# Autodesk Inventor assembly: Gearbox Assembly
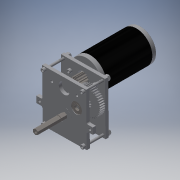
[picture p0: Inventor's stored thumbnail of the model, 180x180]
Saved by Autodesk Inventor 2018 (Build 220112000, 112)
## iProperties
Created: 2019-01-19
Part Number: Gearbox Assembly
Description: STEP AP203
Document SubType Name: Assembly
Designer: maste
Sending System: SolidWorks 2018
Preprocessor: SwSTEP 2.0
Title: Gear_Box.STEP
Revision Number: ANY
## Documents named in this file (17)
- C:\Users\s-2512711\Desktop\Github\2019CAD\Drivebase but Calvin is a mad man\Gearbox Assembly.iam
- C:\Users\s-2512711\Desktop\Github\2019CAD\Drivebase but Calvin is a mad man\CIM_Motor_217-2000.ipt
- C:\Users\s-2512711\Desktop\Github\2019CAD\Drivebase but Calvin is a mad man\12t_Steel_Spur_Gear_20_DP_CIM_Motor_217-3099.ipt
- C:\Users\s-2512711\Desktop\Github\2019CAD\Drivebase but Calvin is a mad man\14t_Steel_Spur_Gear_20_DP_3_8_Hex_Bore_217-3100.step.ipt
- C:\Users\s-2512711\Desktop\Github\2019CAD\Drivebase but Calvin is a mad man\40t_Aluminum_Spur_Gear_20_DP_3_8_Hex_Bore_217-2707.step.ipt
- C:\Users\s-2512711\Desktop\Github\2019CAD\Drivebase but Calvin is a mad man\Not Tiberculosis TB Hex Shaft.ipt
- C:\Users\s-2512711\Desktop\Github\2019CAD\Drivebase but Calvin is a mad man\Gearbox Plate.ipt
- C:\Users\s-2512711\Desktop\Github\2019CAD\Drivebase but Calvin is a mad man\Gearbox Plate V2.ipt
- C:\Users\s-2512711\Desktop\Github\2019CAD\Drivebase but Calvin is a mad man\40t_Aluminum_Spur_Gear_20_DP_3_8_Hex_Bore_217-2707.ipt
- C:\Users\s-2512711\Desktop\Github\2019CAD\Drivebase but Calvin is a mad man\0_375_Hex_ID_x_1_125_OD_x_0_313_WD_Flanged_Bearing_217-2735.ipt
- C:\Users\s-2512711\Desktop\Github\2019CAD\Drivebase but Calvin is a mad man\375 Hex Output Shaft.ipt
- C:\Users\s-2512711\Desktop\Github\2019CAD\Drivebase but Calvin is a mad man\250x1000 dowel.ipt
- C:\Users\s-2512711\Desktop\Github\2019CAD\Drivebase but Calvin is a mad man\92196A272_18-8 STAINLESS STEEL SOCKET HEAD CAP SCREW.ipt
- C:\Users\s-2512711\Desktop\Github\2019CAD\Drivebase but Calvin is a mad man\0.125 0.375 Spacer.ipt
- C:\Users\s-2512711\Desktop\Github\2019CAD\Drivebase but Calvin is a mad man\92196A253_18-8 STAINLESS STEEL SOCKET HEAD CAP SCREW.ipt
- C:\Users\s-2512711\Desktop\Github\2019CAD\Drivebase but Calvin is a mad man\91831A011_TYPE 18-8 STAINLESS STL NYLON-INSERT LOCKNUT.ipt
- C:\Users\s-2512711\Desktop\Github\2019CAD\Drivebase but Calvin is a mad man\10_25mm_3_8_ThunderHex_ID_x_0_875_OD_x_0_280_WD_Flanged_Bearing_217-5829 (1).ipt
## Components (25 placed, 18 different names)
1. CIM_Motor_217-2000.step_1 — Mate:1, Mate:24, Mate:25, Mate:26, Mate:74
2. 12t_Aluminum_Spur_Gear_20_DP_CIM_Motor_217-2614.step_2 — Mate:1, Mate:74
3. 14t_Steel_Spur_Gear_20_DP_3_8_Hex_Bore_217-3100.step_3 — Mate:17, Mate:18, Mate:19
4. 40t_Aluminum_Spur_Gear_20_DP_3_8_Hex_Bore_217-2707.step_4 — Mate:15, Mate:16, Mate:17, Mate:56
5. 10_25mm_3_8_ThunderHex_ID_x_0_875_OD_x_0_280_WD_Flanged_Bearing_217-5829.step_8
6. 10_25mm_3_8_ThunderHex_ID_x_0_875_OD_x_0_280_WD_Flanged_Bearing_217-5829.step_11
7. Not Tiberculosis TB Hex Shaft:2 — Mate:15, Mate:16, Mate:18, Mate:19, Mate:54, Mate:55
8. Gearbox Plate V2:1 — Mate:24, Mate:25, Mate:26, Flush:1, Flush:2, Mate:49, Mate:50, Mate:51, Mate:52, Mate:66, Mate:67, Mate:68, Mate:69
9. 10_25mm_3_8_ThunderHex_ID_x_0_875_OD_x_0_280_WD_Flanged_Bearing_217-5829 (1):3
10. 40t_Aluminum_Spur_Gear_20_DP_3_8_Hex_Bore_217-2707:1 — Mate:35, Flush:3, Flush:4
11. 0_375_Hex_ID_x_1_125_OD_x_0_313_WD_Flanged_Bearing_217-2735:1 — Mate:33, Mate:34, Mate:35, Flush:3, Flush:4
12. Gearbox Plate:1 — Flush:1, Flush:2, Mate:33, Mate:34, Mate:58, Mate:59, Mate:60, Mate:61, Mate:62, Mate:63, Mate:64, Mate:65
13. 375 Hex Output Shaft:1 — Mate:36, Mate:37
14. 250x1000 dowel:1 — Mate:36, Mate:37
15. 92196A272_18-8 STAINLESS STEEL SOCKET HEAD CAP SCREW:1 — Mate:51, Mate:52
16. 92196A272_18-8 STAINLESS STEEL SOCKET HEAD CAP SCREW:2 — Mate:49, Mate:50
17. 0.125 0.375 Spacer:1 — Mate:54, Mate:55, Mate:56
18. 92196A253_18-8 STAINLESS STEEL SOCKET HEAD CAP SCREW:1 — Mate:60, Mate:62, Mate:73
19. 92196A253_18-8 STAINLESS STEEL SOCKET HEAD CAP SCREW:2 — Mate:61, Mate:63, Mate:70
20. 92196A253_18-8 STAINLESS STEEL SOCKET HEAD CAP SCREW:3 — Mate:59, Mate:65, Mate:71
21. 92196A253_18-8 STAINLESS STEEL SOCKET HEAD CAP SCREW:4 — Mate:58, Mate:64, Mate:72
22. 91831A011_TYPE 18-8 STAINLESS STL NYLON-INSERT LOCKNUT:1 — Mate:68, Mate:71
23. 91831A011_TYPE 18-8 STAINLESS STL NYLON-INSERT LOCKNUT:2 — Mate:67, Mate:72
24. 91831A011_TYPE 18-8 STAINLESS STL NYLON-INSERT LOCKNUT:3 — Mate:66, Mate:73
25. 91831A011_TYPE 18-8 STAINLESS STL NYLON-INSERT LOCKNUT:4 — Mate:69, Mate:70
## Relationships (54: Mate 50, Flush 4)
- Mate:1: CIM_Motor_217-2000.step_1 ↔ 12t_Aluminum_Spur_Gear_20_DP_CIM_Motor_217-2614.step_2
- [Mate]: 10_25mm_3_8_ThunderHex_ID_x_0_875_OD_x_0_280_WD_Flanged_Bearing_217-5829.step_11 ↔ Not Tiberculosis TB Hex Shaft:2
- [Mate]: 10_25mm_3_8_ThunderHex_ID_x_0_875_OD_x_0_280_WD_Flanged_Bearing_217-5829.step_11 ↔ Not Tiberculosis TB Hex Shaft:2
- Mate:15: 40t_Aluminum_Spur_Gear_20_DP_3_8_Hex_Bore_217-2707.step_4 ↔ Not Tiberculosis TB Hex Shaft:2
- Mate:16: 40t_Aluminum_Spur_Gear_20_DP_3_8_Hex_Bore_217-2707.step_4 ↔ Not Tiberculosis TB Hex Shaft:2
- Mate:17: 14t_Steel_Spur_Gear_20_DP_3_8_Hex_Bore_217-3100.step_3 ↔ 40t_Aluminum_Spur_Gear_20_DP_3_8_Hex_Bore_217-2707.step_4
- Mate:18: 14t_Steel_Spur_Gear_20_DP_3_8_Hex_Bore_217-3100.step_3 ↔ Not Tiberculosis TB Hex Shaft:2
- Mate:19: 14t_Steel_Spur_Gear_20_DP_3_8_Hex_Bore_217-3100.step_3 ↔ Not Tiberculosis TB Hex Shaft:2
- [Mate]: 10_25mm_3_8_ThunderHex_ID_x_0_875_OD_x_0_280_WD_Flanged_Bearing_217-5829.step_11 ↔ Gearbox Plate V2:1
- [Mate]: 10_25mm_3_8_ThunderHex_ID_x_0_875_OD_x_0_280_WD_Flanged_Bearing_217-5829.step_11 ↔ Gearbox Plate V2:1
- Mate:24: CIM_Motor_217-2000.step_1 ↔ Gearbox Plate V2:1
- Mate:25: CIM_Motor_217-2000.step_1 ↔ Gearbox Plate V2:1
- Mate:26: CIM_Motor_217-2000.step_1 ↔ Gearbox Plate V2:1
- [Mate]: 10_25mm_3_8_ThunderHex_ID_x_0_875_OD_x_0_280_WD_Flanged_Bearing_217-5829.step_8 ↔ Not Tiberculosis TB Hex Shaft:2
- [Mate]: Gearbox Plate V2:1 ↔ 10_25mm_3_8_ThunderHex_ID_x_0_875_OD_x_0_280_WD_Flanged_Bearing_217-5829 (1):3
- [Mate]: Gearbox Plate V2:1 ↔ 10_25mm_3_8_ThunderHex_ID_x_0_875_OD_x_0_280_WD_Flanged_Bearing_217-5829 (1):3
- Flush:1: Gearbox Plate V2:1 ↔ Gearbox Plate:1
- Flush:2: Gearbox Plate V2:1 ↔ Gearbox Plate:1
- Mate:33: 0_375_Hex_ID_x_1_125_OD_x_0_313_WD_Flanged_Bearing_217-2735:1 ↔ Gearbox Plate:1
- Mate:34: 0_375_Hex_ID_x_1_125_OD_x_0_313_WD_Flanged_Bearing_217-2735:1 ↔ Gearbox Plate:1
- Mate:35: 40t_Aluminum_Spur_Gear_20_DP_3_8_Hex_Bore_217-2707:1 ↔ 0_375_Hex_ID_x_1_125_OD_x_0_313_WD_Flanged_Bearing_217-2735:1
- Flush:3: 40t_Aluminum_Spur_Gear_20_DP_3_8_Hex_Bore_217-2707:1 ↔ 0_375_Hex_ID_x_1_125_OD_x_0_313_WD_Flanged_Bearing_217-2735:1
- Flush:4: 40t_Aluminum_Spur_Gear_20_DP_3_8_Hex_Bore_217-2707:1 ↔ 0_375_Hex_ID_x_1_125_OD_x_0_313_WD_Flanged_Bearing_217-2735:1
- Mate:36: 375 Hex Output Shaft:1 ↔ 250x1000 dowel:1
- Mate:37: 375 Hex Output Shaft:1 ↔ 250x1000 dowel:1
- [Mate]: 10_25mm_3_8_ThunderHex_ID_x_0_875_OD_x_0_280_WD_Flanged_Bearing_217-5829 (1):3 ↔ 375 Hex Output Shaft:1
- [Mate]: 10_25mm_3_8_ThunderHex_ID_x_0_875_OD_x_0_280_WD_Flanged_Bearing_217-5829 (1):3 ↔ 375 Hex Output Shaft:1
- [Mate]: 10_25mm_3_8_ThunderHex_ID_x_0_875_OD_x_0_280_WD_Flanged_Bearing_217-5829.step_8 ↔ Gearbox Plate:1
- Mate:49: Gearbox Plate V2:1 ↔ 92196A272_18-8 STAINLESS STEEL SOCKET HEAD CAP SCREW:2
- Mate:50: Gearbox Plate V2:1 ↔ 92196A272_18-8 STAINLESS STEEL SOCKET HEAD CAP SCREW:2
- Mate:51: Gearbox Plate V2:1 ↔ 92196A272_18-8 STAINLESS STEEL SOCKET HEAD CAP SCREW:1
- Mate:52: Gearbox Plate V2:1 ↔ 92196A272_18-8 STAINLESS STEEL SOCKET HEAD CAP SCREW:1
- [Mate]: 10_25mm_3_8_ThunderHex_ID_x_0_875_OD_x_0_280_WD_Flanged_Bearing_217-5829.step_11 ↔ 0.125 0.375 Spacer:1
- Mate:54: Not Tiberculosis TB Hex Shaft:2 ↔ 0.125 0.375 Spacer:1
- Mate:55: Not Tiberculosis TB Hex Shaft:2 ↔ 0.125 0.375 Spacer:1
- Mate:56: 40t_Aluminum_Spur_Gear_20_DP_3_8_Hex_Bore_217-2707.step_4 ↔ 0.125 0.375 Spacer:1
- [Mate]: 14t_Steel_Spur_Gear_20_DP_3_8_Hex_Bore_217-3100.step_3 ↔ 10_25mm_3_8_ThunderHex_ID_x_0_875_OD_x_0_280_WD_Flanged_Bearing_217-5829.step_8
- Mate:58: Gearbox Plate:1 ↔ 92196A253_18-8 STAINLESS STEEL SOCKET HEAD CAP SCREW:4
- Mate:59: Gearbox Plate:1 ↔ 92196A253_18-8 STAINLESS STEEL SOCKET HEAD CAP SCREW:3
- Mate:60: Gearbox Plate:1 ↔ 92196A253_18-8 STAINLESS STEEL SOCKET HEAD CAP SCREW:1
- Mate:61: Gearbox Plate:1 ↔ 92196A253_18-8 STAINLESS STEEL SOCKET HEAD CAP SCREW:2
- Mate:62: Gearbox Plate:1 ↔ 92196A253_18-8 STAINLESS STEEL SOCKET HEAD CAP SCREW:1
- Mate:63: Gearbox Plate:1 ↔ 92196A253_18-8 STAINLESS STEEL SOCKET HEAD CAP SCREW:2
- Mate:64: Gearbox Plate:1 ↔ 92196A253_18-8 STAINLESS STEEL SOCKET HEAD CAP SCREW:4
- Mate:65: Gearbox Plate:1 ↔ 92196A253_18-8 STAINLESS STEEL SOCKET HEAD CAP SCREW:3
- Mate:66: Gearbox Plate V2:1 ↔ 91831A011_TYPE 18-8 STAINLESS STL NYLON-INSERT LOCKNUT:3
- Mate:67: Gearbox Plate V2:1 ↔ 91831A011_TYPE 18-8 STAINLESS STL NYLON-INSERT LOCKNUT:2
- Mate:68: Gearbox Plate V2:1 ↔ 91831A011_TYPE 18-8 STAINLESS STL NYLON-INSERT LOCKNUT:1
- Mate:69: Gearbox Plate V2:1 ↔ 91831A011_TYPE 18-8 STAINLESS STL NYLON-INSERT LOCKNUT:4
- Mate:70: 92196A253_18-8 STAINLESS STEEL SOCKET HEAD CAP SCREW:2 ↔ 91831A011_TYPE 18-8 STAINLESS STL NYLON-INSERT LOCKNUT:4
- Mate:71: 92196A253_18-8 STAINLESS STEEL SOCKET HEAD CAP SCREW:3 ↔ 91831A011_TYPE 18-8 STAINLESS STL NYLON-INSERT LOCKNUT:1
- Mate:72: 92196A253_18-8 STAINLESS STEEL SOCKET HEAD CAP SCREW:4 ↔ 91831A011_TYPE 18-8 STAINLESS STL NYLON-INSERT LOCKNUT:2
- Mate:73: 92196A253_18-8 STAINLESS STEEL SOCKET HEAD CAP SCREW:1 ↔ 91831A011_TYPE 18-8 STAINLESS STL NYLON-INSERT LOCKNUT:3
- Mate:74: CIM_Motor_217-2000.step_1 ↔ 12t_Aluminum_Spur_Gear_20_DP_CIM_Motor_217-2614.step_2
